# Autodesk Inventor assembly: Harmonic Mount Complete Assembly
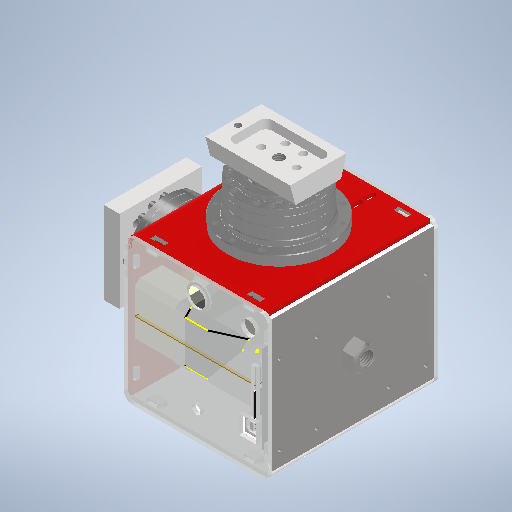
[picture p0: Inventor's stored thumbnail of the model, 512x512]
Saved by Autodesk Inventor 2025 (Build 290162000, 162)
## iProperties
Created: 2025-08-10
Part Number: Harmonic Mount Complete Assembly
Document SubType Name: Assembly
Designer: yshis
Author: yshis
## Documents named in this file (17)
- C:\Users\yshis\Documents\Harmonic Drive Mount\Harmonic Mount Complete Assembly.iam
- C:\Users\yshis\Documents\Harmonic Drive Mount\Harmonic Mount Box Assembly.iam
- C:\Users\yshis\Documents\Harmonic Drive Mount\CSF-17-XXX-2UH.iam
- C:\Users\yshis\Documents\Harmonic Drive Mount\Shaft 8mm.ipt
- C:\Users\yshis\Documents\Harmonic Drive Mount\GT2-60T-5BW-Bore8.ipt
- C:\Users\yshis\Documents\Harmonic Drive Mount\Bearing.ipt
- C:\Users\yshis\Documents\Harmonic Drive Mount\Base for NEMA17.ipt
- C:\Users\yshis\Documents\Harmonic Drive Mount\NEMA_17_42x60.ipt
- C:\Users\yshis\Documents\Harmonic Drive Mount\GT2_20T_dzino.ipt
- C:\Users\yshis\Documents\Harmonic Drive Mount\FYSETC E4 Board.ipt
- C:\Users\yshis\Documents\Harmonic Drive Mount\Cover-USB side.ipt
- C:\Users\yshis\Documents\Harmonic Drive Mount\Cover side-2.ipt
- C:\Users\yshis\Documents\Harmonic Drive Mount\Wedge-Dove tail.ipt
- C:\Users\yshis\Documents\Harmonic Drive Mount\Adapter plate for tube dovetail bracket.ipt
- C:\Users\yshis\Documents\Harmonic Drive Mount\Grease retainer disk.ipt
- C:\Users\yshis\Documents\Harmonic Drive Mount\Pulley Bearing Support.-3.ipt
- C:\Users\yshis\Documents\Inventor\Content Center Files\R2025\en-US\BS EN ISO 7045 H\EN ISO 7045 - M4 x 16 - 4.8 - H(1).ipt
## Components (25 placed, 16 different names)
1. Harmonic Mount Box Assembly:1 [sub-assembly] — Mate:1, Mate:2, Mate:3, Mate:4, Mate:5, Mate:6, Mate:10, Mate:12, Mate:26, Mate:27, Angle:1, Angle:2, Flush:3, Flush:5, Flush:7, Flush:8, Mate:42, Angle:4, Mate:44, Mate:45, Mate:46, Flush:14, Flush:15, Mate:47, Flush:16, Flush:17, Mate:54, Mate:55, Mate:56, Mate:57, Mate:58, Mate:59, Mate:60, Mate:61, Mate:62, Mate:63
2. CSF-17-XXX-2UH:1 [sub-assembly] — Mate:1, Mate:2, Mate:6, Mate:8, Mate:51, Mate:52, Mate:53
3. CSF-17-XXX-2UH:2 [sub-assembly] — Mate:3, Mate:4, Mate:5, Mate:9, Mate:48, Mate:49, Mate:50
4. Shaft 8mm:1 — Mate:9, Mate:11, Mate:24, Flush:2
5. Shaft 8mm:2 — Mate:8, Mate:13, Mate:22, Flush:1
6. GT2-60T-5BW-Bore8:1 — Mate:10, Mate:11
7. GT2-60T-5BW-Bore8:2 — Mate:12, Mate:13
8. Bearing:1 — Mate:24, Flush:2, Mate:66, Mate:67
9. Bearing:2 — Mate:22, Flush:1, Mate:64, Mate:65
10. Base for NEMA17:1 — Mate:26, Mate:28, Mate:29, Mate:30, Angle:2, Flush:7, Mate:38, Flush:12, Flush:13
11. Base for NEMA17:2 — Mate:27, Mate:31, Mate:32, Mate:33, Angle:1, Flush:8, Mate:68, Mate:69, Angle:5, Angle:6
12. NEMA_17_42x60:1 — Angle:4, Mate:38, Mate:41, Flush:10, Flush:12, Mate:43, Flush:13
13. GT2_20T_dzino:1 — Mate:41, Flush:10
14. GT2_20T_dzino:2 — Mate:70
15. FYSETC E4 Board:1 — Mate:42, Mate:44, Mate:45
16. Cover-USB side:1 — Mate:46, Flush:14, Flush:15
17. Cover side-2:1 — Mate:47, Flush:16, Flush:17
18. Wedge-Dove tail:1 — Mate:48, Mate:49, Mate:50
19. Adapter plate for tube dovetail bracket:1 — Mate:51, Mate:52, Mate:53
20. Grease retainer disk:1 — Mate:54, Mate:55
21. Grease retainer disk:2 — Mate:56, Mate:57
22. Pulley Bearing Support.-3:1 — Mate:58, Mate:60, Mate:62, Mate:66, Mate:67, Insert:1
23. Pulley Bearing Support.-3:2 — Mate:59, Mate:61, Mate:63, Mate:64, Mate:65
24. BS EN ISO 7045 H - Metric M4 x 16 - 4.8 - H:1 — Insert:1
25. NEMA_17_42x60:2 — Mate:68, Mate:69, Angle:5, Angle:6, Mate:70
## Relationships (74: Mate 53, Flush 15, Angle 5, Insert 1)
- Mate:1: Harmonic Mount Box Assembly:1 ↔ CSF-17-XXX-2UH:1
- Mate:2: Harmonic Mount Box Assembly:1 ↔ CSF-17-XXX-2UH:1
- Mate:3: Harmonic Mount Box Assembly:1 ↔ CSF-17-XXX-2UH:2
- Mate:4: Harmonic Mount Box Assembly:1 ↔ CSF-17-XXX-2UH:2
- Mate:5: Harmonic Mount Box Assembly:1 ↔ CSF-17-XXX-2UH:2
- Mate:6: Harmonic Mount Box Assembly:1 ↔ CSF-17-XXX-2UH:1
- Mate:8: CSF-17-XXX-2UH:1 ↔ Shaft 8mm:2
- Mate:9: CSF-17-XXX-2UH:2 ↔ Shaft 8mm:1
- Mate:10 (5 mm): Harmonic Mount Box Assembly:1 ↔ GT2-60T-5BW-Bore8:1
- Mate:11: Shaft 8mm:1 ↔ GT2-60T-5BW-Bore8:1
- Mate:12 (5 mm): Harmonic Mount Box Assembly:1 ↔ GT2-60T-5BW-Bore8:2
- Mate:13: Shaft 8mm:2 ↔ GT2-60T-5BW-Bore8:2
- Mate:22: Shaft 8mm:2 ↔ Bearing:2
- Flush:1 (-1 mm): Shaft 8mm:2 ↔ Bearing:2
- Mate:24: Shaft 8mm:1 ↔ Bearing:1
- Flush:2 (-1 mm): Shaft 8mm:1 ↔ Bearing:1
- Mate:26: Harmonic Mount Box Assembly:1 ↔ Base for NEMA17:1
- Mate:27: Harmonic Mount Box Assembly:1 ↔ Base for NEMA17:2
- Mate:28: Base for NEMA17:1
- Mate:29: Base for NEMA17:1
- Mate:30: Base for NEMA17:1
- Mate:31: Base for NEMA17:2
- Mate:32: Base for NEMA17:2
- Mate:33: Base for NEMA17:2
- Angle:1 (0 deg): Harmonic Mount Box Assembly:1 ↔ Base for NEMA17:2
- Angle:2 (0 deg): Harmonic Mount Box Assembly:1 ↔ Base for NEMA17:1
- Flush:3 (-54 mm): Harmonic Mount Box Assembly:1
- Flush:4
- Flush:5 (-54 mm): Harmonic Mount Box Assembly:1
- Flush:6
- Flush:7 (-2 mm): Harmonic Mount Box Assembly:1 ↔ Base for NEMA17:1
- Flush:8 (-2 mm): Harmonic Mount Box Assembly:1 ↔ Base for NEMA17:2
- Angle:4 (0 deg): Harmonic Mount Box Assembly:1 ↔ NEMA_17_42x60:1
- Mate:38: Base for NEMA17:1 ↔ NEMA_17_42x60:1
- Mate:41: NEMA_17_42x60:1 ↔ GT2_20T_dzino:1
- Flush:10: NEMA_17_42x60:1 ↔ GT2_20T_dzino:1
- Mate:42 (5 mm): Harmonic Mount Box Assembly:1 ↔ FYSETC E4 Board:1
- Flush:12: Base for NEMA17:1 ↔ NEMA_17_42x60:1
- Mate:43: NEMA_17_42x60:1
- Flush:13: Base for NEMA17:1 ↔ NEMA_17_42x60:1
- Mate:44: Harmonic Mount Box Assembly:1 ↔ FYSETC E4 Board:1
- Mate:45: Harmonic Mount Box Assembly:1 ↔ FYSETC E4 Board:1
- Mate:46: Harmonic Mount Box Assembly:1 ↔ Cover-USB side:1
- Flush:14: Harmonic Mount Box Assembly:1 ↔ Cover-USB side:1
- Flush:15: Harmonic Mount Box Assembly:1 ↔ Cover-USB side:1
- Mate:47: Harmonic Mount Box Assembly:1 ↔ Cover side-2:1
- Flush:16: Harmonic Mount Box Assembly:1 ↔ Cover side-2:1
- Flush:17: Harmonic Mount Box Assembly:1 ↔ Cover side-2:1
- Mate:48: CSF-17-XXX-2UH:2 ↔ Wedge-Dove tail:1
- Mate:49: CSF-17-XXX-2UH:2 ↔ Wedge-Dove tail:1
- Mate:50: CSF-17-XXX-2UH:2 ↔ Wedge-Dove tail:1
- Mate:51: CSF-17-XXX-2UH:1 ↔ Adapter plate for tube dovetail bracket:1
- Mate:52: CSF-17-XXX-2UH:1 ↔ Adapter plate for tube dovetail bracket:1
- Mate:53: CSF-17-XXX-2UH:1 ↔ Adapter plate for tube dovetail bracket:1
- Mate:54: Harmonic Mount Box Assembly:1 ↔ Grease retainer disk:1
- Mate:55: Harmonic Mount Box Assembly:1 ↔ Grease retainer disk:1
- Mate:56: Harmonic Mount Box Assembly:1 ↔ Grease retainer disk:2
- Mate:57: Harmonic Mount Box Assembly:1 ↔ Grease retainer disk:2
- Mate:58: Harmonic Mount Box Assembly:1 ↔ Pulley Bearing Support.-3:1
- Mate:59: Harmonic Mount Box Assembly:1 ↔ Pulley Bearing Support.-3:2
- Mate:60: Harmonic Mount Box Assembly:1 ↔ Pulley Bearing Support.-3:1
- Mate:61: Harmonic Mount Box Assembly:1 ↔ Pulley Bearing Support.-3:2
- Mate:62: Harmonic Mount Box Assembly:1 ↔ Pulley Bearing Support.-3:1
- Mate:63: Harmonic Mount Box Assembly:1 ↔ Pulley Bearing Support.-3:2
- Mate:64: Bearing:2 ↔ Pulley Bearing Support.-3:2
- Mate:65: Bearing:2 ↔ Pulley Bearing Support.-3:2
- Mate:66: Bearing:1 ↔ Pulley Bearing Support.-3:1
- Mate:67: Bearing:1 ↔ Pulley Bearing Support.-3:1
- Insert:1: Pulley Bearing Support.-3:1 ↔ BS EN ISO 7045 H - Metric M4 x 16 - 4.8 - H:1
- Mate:68: Base for NEMA17:2 ↔ NEMA_17_42x60:2
- Mate:69: Base for NEMA17:2 ↔ NEMA_17_42x60:2
- Angle:5 (0 deg): Base for NEMA17:2 ↔ NEMA_17_42x60:2
- Angle:6 (0 deg): Base for NEMA17:2 ↔ NEMA_17_42x60:2
- Mate:70: GT2_20T_dzino:2 ↔ NEMA_17_42x60:2
